# Autodesk Inventor assembly: Передача с помощью зубчатых ремней
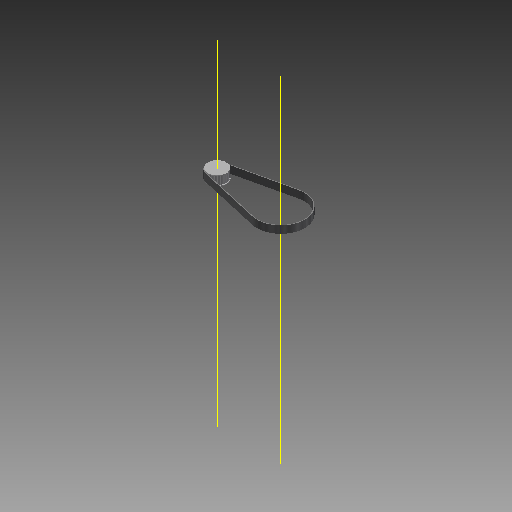
[picture p0: Inventor's stored thumbnail of the model, 512x512]
Saved by Autodesk Inventor 2019.1 (Build 231200000, 200)
## iProperties
ClientObjectVersion: 1
Created: 2018-10-15
Part Number: Передача с помощью зубчатых ремней
Document SubType Name: Assembly
Designer: Олег
Author: Олег
## Documents named in this file (3)
- C:\Users\Олег\OneDrive\Общая\NoSpace 2.0\Манипулятор\Блок подъёма первога звена\Мастер проектирования\Передача с помощью зубчатых ремней4.iam
- C:\Users\Олег\OneDrive\Общая\NoSpace 2.0\Манипулятор\Блок подъёма первога звена\Мастер проектирования\Зубчатый ремень4.ipt
- C:\Users\Олег\OneDrive\Общая\NoSpace 2.0\Манипулятор\Блок подъёма первога звена\Мастер проектирования\Синхронный шкив23.ipt
## Components (2 placed, 2 different names)
1. Зубчатый ремень:1 — Заподлицо:1, Совмещение:1, Совмещение:2
2. Синхронный шкив2:1 — Заподлицо:1, Совмещение:1, Совмещение:2
## Relationships (3: Mate 2, Flush 1)
- Заподлицо:1 [Flush]: Зубчатый ремень:1 ↔ Синхронный шкив2:1
- Совмещение:1 [Mate]: Зубчатый ремень:1 ↔ Синхронный шкив2:1
- Совмещение:2 [Mate]: Зубчатый ремень:1 ↔ Синхронный шкив2:1
